# Autodesk Inventor assembly: UBG-Compute Layer
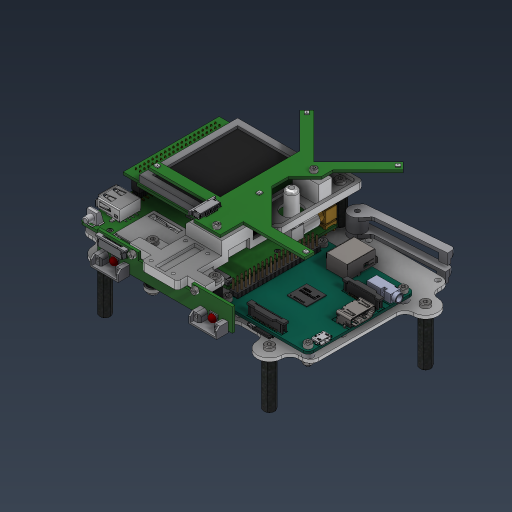
[picture p0: Inventor's stored thumbnail of the model, 512x512]
Saved by Autodesk Inventor 2023.1 (Build 271208000, 208)
## iProperties
Part Number: UBG-Compute Layer
Material: Generisch
Document SubType Name: Assembly
Designer: rYan
Mass: 227.724 g
Surface Area: 1110.42 cm^2
Volume: 92.4651 cm^3
Density: 2.46281 g/cm^3
Author: rYan
## Documents named in this file (14)
- D:\TIGERsGIT\Hardware\mechanik\2020\Inventor\Robot\Electronics\UBG-Compute Layer.iam
- D:\TIGERsGIT\Hardware\mechanik\2020\Inventor\Robot\Electronics\Oberplatte.ipt
- D:\TIGERsGIT\Hardware\mechanik\2020\Inventor\Robot\Electronics\MG-Mainboard.iam
- D:\TIGERsGIT\Hardware\mechanik\2019\Inventor\Kaufteile\Abstandsbolzen Typ A.ipt
- D:\TIGERsGIT\Hardware\mechanik\2020\Inventor\Inhaltscenter\de-DE\DIN 7984\DIN 7984 - M3 x 5.ipt
- D:\TIGERsGIT\Hardware\mechanik\2020\Inventor\Robot\Electronics\UBG-Stereokamera.iam
- D:\TIGERsGIT\Hardware\mechanik\2020\Inventor\Purchased Parts\Abstandsbolzen Typ A M3 30mm SW6.ipt
- D:\TIGERsGIT\Hardware\mechanik\2020\Inventor\Inhaltscenter\de-DE\ISO 4762(2)\ISO 4762 - M2 x 6ISO.ipt
- D:\TIGERsGIT\Hardware\mechanik\2020\Inventor\Purchased Parts\Raspberry Pi 3A+.ipt
- D:\TIGERsGIT\Hardware\mechanik\2020\Inventor\Robot\Electronics\Akkusperre.ipt
- D:\TIGERsGIT\Hardware\mechanik\2020\Inventor\Purchased Parts\Spacer M3 3mm.ipt
- D:\TIGERsGIT\Hardware\mechanik\2020\Inventor\Inhaltscenter\de-DE\ISO 4762(1)\DIN EN ISO 4762 - M2,5 x 10.ipt
- D:\TIGERsGIT\Hardware\mechanik\2020\Inventor\Inhaltscenter\de-DE\DIN 934\DIN 934 - M2,5 x 0,45.ipt
- D:\TIGERsGIT\Hardware\mechanik\2020\Inventor\Robot\Electronics\Akkusperre Klein.ipt
## Components (33 placed, 12 different names)
1. Oberplatte:1 — Fluchtend:1, Fluchtend:2, Fluchtend:3, Einfügen:1, Einfügen:2, Einfügen:3, Einfügen:4, Einfügen:5, Einfügen:6, Einfügen:7, Einfügen:8, Einfügen:11, Passend:8, Einfügen:12, Einfügen:13, Einfügen:14, Passend:14, Einfügen:19, Einfügen:20, Einfügen:21, Einfügen:22, Passend:15, Einfügen:23, Einfügen:33, Einfügen:34, Einfügen:35, Einfügen:36, Einfügen:38, Einfügen:39
2. MG-Mainboard:1 [sub-assembly] — Passend:3, Passend:4, Passend:14
3. UBG-Stereokamera:1 [sub-assembly] — Einfügen:11, Passend:8
4. Abstandsbolzen Typ A M3 30mm SW6:1 — Einfügen:4
5. Abstandsbolzen Typ A M3 30mm SW6:2 — Einfügen:3
6. Abstandsbolzen Typ A M3 30mm SW6:3 — Einfügen:2
7. Abstandsbolzen Typ A M3 30mm SW6:4 — Einfügen:1
8. DIN 7984 M3 x 5:1 — Einfügen:5
9. DIN 7984 M3 x 5:2 — Einfügen:6
10. DIN 7984 M3 x 5:3 — Einfügen:7
11. DIN 7984 M3 x 5:4 — Einfügen:8
12. DIN 7984 M3 x 5:5 — Einfügen:14
13. DIN 7984 M3 x 5:6 — Einfügen:13
14. DIN 7984 M3 x 5:7 — Einfügen:12
15. ISO 4762 M2 x 6:1 — Einfügen:21
16. ISO 4762 M2 x 6:2 — Einfügen:20
17. ISO 4762 M2 x 6:3 — Einfügen:19
18. Raspberry Pi 3A+:1 — Einfügen:22, Passend:15, Einfügen:25, Einfügen:26, Einfügen:27, Einfügen:28, Einfügen:29, Einfügen:30, Einfügen:31, Einfügen:32
19. Akkusperre:1 — Einfügen:23, Einfügen:37
20. Spacer M3 3mm:1 — Einfügen:25
21. Spacer M3 3mm:2 — Einfügen:28
22. Spacer M3 3mm:3 — Einfügen:27
23. Spacer M3 3mm:4 — Einfügen:26
24. DIN EN ISO 4762 M2,5 x 10:1 — Einfügen:29
25. DIN EN ISO 4762 M2,5 x 10:2 — Einfügen:30
26. DIN EN ISO 4762 M2,5 x 10:3 — Einfügen:31
27. DIN EN ISO 4762 M2,5 x 10:4 — Einfügen:32
28. DIN 934 - ersetzt durch DIN EN 24032/28673/28674 M2,5:1 — Einfügen:33
29. DIN 934 - ersetzt durch DIN EN 24032/28673/28674 M2,5:2 — Einfügen:34
30. DIN 934 - ersetzt durch DIN EN 24032/28673/28674 M2,5:3 — Einfügen:35
31. DIN 934 - ersetzt durch DIN EN 24032/28673/28674 M2,5:4 — Einfügen:36
32. Akkusperre Klein:1 — Einfügen:37, Einfügen:38
33. DIN 7984 M3 x 5:8 — Einfügen:39
## Relationships (40: Insert 32, Mate 5, Flush 3)
- Fluchtend:1 [Flush]: Oberplatte:1
- Fluchtend:2 [Flush]: Oberplatte:1
- Fluchtend:3 [Flush]: Oberplatte:1
- Einfügen:1 [Insert]: Oberplatte:1 ↔ Abstandsbolzen Typ A M3 30mm SW6:4
- Einfügen:2 [Insert]: Oberplatte:1 ↔ Abstandsbolzen Typ A M3 30mm SW6:3
- Einfügen:3 [Insert]: Oberplatte:1 ↔ Abstandsbolzen Typ A M3 30mm SW6:2
- Einfügen:4 [Insert]: Oberplatte:1 ↔ Abstandsbolzen Typ A M3 30mm SW6:1
- Einfügen:5 [Insert]: Oberplatte:1 ↔ DIN 7984 M3 x 5:1
- Einfügen:6 [Insert]: Oberplatte:1 ↔ DIN 7984 M3 x 5:2
- Einfügen:7 [Insert]: Oberplatte:1 ↔ DIN 7984 M3 x 5:3
- Einfügen:8 [Insert]: Oberplatte:1 ↔ DIN 7984 M3 x 5:4
- Passend:3 [Mate]: MG-Mainboard:1
- Passend:4 [Mate]: MG-Mainboard:1
- Einfügen:11 [Insert]: Oberplatte:1 ↔ UBG-Stereokamera:1
- Passend:8 [Mate]: Oberplatte:1 ↔ UBG-Stereokamera:1
- Einfügen:12 [Insert]: Oberplatte:1 ↔ DIN 7984 M3 x 5:7
- Einfügen:13 [Insert]: Oberplatte:1 ↔ DIN 7984 M3 x 5:6
- Einfügen:14 [Insert]: Oberplatte:1 ↔ DIN 7984 M3 x 5:5
- Passend:14 [Mate]: Oberplatte:1 ↔ MG-Mainboard:1
- Einfügen:19 [Insert]: Oberplatte:1 ↔ ISO 4762 M2 x 6:3
- Einfügen:20 [Insert]: Oberplatte:1 ↔ ISO 4762 M2 x 6:2
- Einfügen:21 [Insert]: Oberplatte:1 ↔ ISO 4762 M2 x 6:1
- Einfügen:22 [Insert] (3 mm): Oberplatte:1 ↔ Raspberry Pi 3A+:1
- Passend:15 [Mate]: Oberplatte:1 ↔ Raspberry Pi 3A+:1
- Einfügen:23 [Insert]: Oberplatte:1 ↔ Akkusperre:1
- Einfügen:25 [Insert]: Raspberry Pi 3A+:1 ↔ Spacer M3 3mm:1
- Einfügen:26 [Insert]: Raspberry Pi 3A+:1 ↔ Spacer M3 3mm:4
- Einfügen:27 [Insert]: Raspberry Pi 3A+:1 ↔ Spacer M3 3mm:3
- Einfügen:28 [Insert]: Raspberry Pi 3A+:1 ↔ Spacer M3 3mm:2
- Einfügen:29 [Insert]: Raspberry Pi 3A+:1 ↔ DIN EN ISO 4762 M2,5 x 10:1
- Einfügen:30 [Insert]: Raspberry Pi 3A+:1 ↔ DIN EN ISO 4762 M2,5 x 10:2
- Einfügen:31 [Insert]: Raspberry Pi 3A+:1 ↔ DIN EN ISO 4762 M2,5 x 10:3
- Einfügen:32 [Insert]: Raspberry Pi 3A+:1 ↔ DIN EN ISO 4762 M2,5 x 10:4
- Einfügen:33 [Insert]: Oberplatte:1 ↔ DIN 934 - ersetzt durch DIN EN 24032/28673/28674 M2,5:1
- Einfügen:34 [Insert]: Oberplatte:1 ↔ DIN 934 - ersetzt durch DIN EN 24032/28673/28674 M2,5:2
- Einfügen:35 [Insert]: Oberplatte:1 ↔ DIN 934 - ersetzt durch DIN EN 24032/28673/28674 M2,5:3
- Einfügen:36 [Insert]: Oberplatte:1 ↔ DIN 934 - ersetzt durch DIN EN 24032/28673/28674 M2,5:4
- Einfügen:37 [Insert]: Akkusperre:1 ↔ Akkusperre Klein:1
- Einfügen:38 [Insert]: Oberplatte:1 ↔ Akkusperre Klein:1
- Einfügen:39 [Insert]: Oberplatte:1 ↔ DIN 7984 M3 x 5:8
